# Autodesk Inventor assembly: BODY
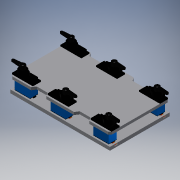
[picture p0: Inventor's stored thumbnail of the model, 180x180]
Saved by Autodesk Inventor 2017 (Build 210142000, 142)
## iProperties
Created: 2017-09-24
Part Number: BODY
Document SubType Name: Assembly
Designer: Alexander Miller
Author: Alexander Miller
## Documents named in this file (4)
- X:\Alex\Documents\Git\HeRo-Mini\Hardware\BODY.iam
- X:\Alex\Documents\Git\HeRo-Mini\Hardware\BODY_BOTTOM.ipt
- X:\Alex\Documents\Git\HeRo-Mini\Hardware\BODY_TOP.ipt
- X:\Alex\Documents\Git\HeRo-Mini\Hardware\SERVO.iam
## Components (8 placed, 3 different names)
1. BODY_BOTTOM:1 — Rigid:8, Rigid:9, Rigid:10, Rigid:11, Rigid:12, Rigid:13
2. BODY_TOP:1 — Rigid:7
3. SERVO:1 [sub-assembly] — Rigid:7, Rigid:13
4. SERVO:2 [sub-assembly] — Rigid:12
5. SERVO:3 [sub-assembly] — Rigid:11
6. SERVO:4 [sub-assembly] — Rigid:10
7. SERVO:5 [sub-assembly] — Rigid:9
8. SERVO:6 [sub-assembly] — Rigid:8
## Relationships (7: WeldJoint 7)
- Rigid:7 [WeldJoint]: BODY_TOP:1 ↔ SERVO:1
- Rigid:8 [WeldJoint]: BODY_BOTTOM:1 ↔ SERVO:6
- Rigid:9 [WeldJoint]: BODY_BOTTOM:1 ↔ SERVO:5
- Rigid:10 [WeldJoint]: BODY_BOTTOM:1 ↔ SERVO:4
- Rigid:11 [WeldJoint]: BODY_BOTTOM:1 ↔ SERVO:3
- Rigid:12 [WeldJoint]: BODY_BOTTOM:1 ↔ SERVO:2
- Rigid:13 [WeldJoint]: BODY_BOTTOM:1 ↔ SERVO:1
